# Autodesk Inventor assembly: White Knight
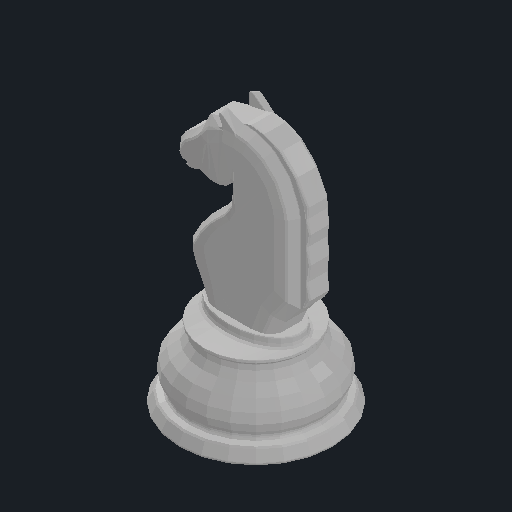
[picture p0: Inventor's stored thumbnail of the model, 512x512]
Saved by Autodesk Inventor 2026 (Build 300175000, 175)
## iProperties
Created: 2025-04-16
Part Number: White Knight
Document SubType Name: Assembly
Designer: ckyiu
Author: ckyiu
## Documents named in this file (3)
- F:\Chessboard-Design\Design\Core\Chess Pieces\Black Knight.iam
- F:\Chessboard-Design\Design\Core\Chess Pieces\Parts\White Knight.ipt
- F:\Chessboard-Design\Design\My-Inventor-Parts\Hardware\(9.5mm diameter 1.6mm height) 5862K143_Neodymium Magnet.ipt
## Components (2 placed, 2 different names)
1. White Knight:1 — Insert:1
2. (9.5mm diameter 1.6mm height) 5862K143_Neodymium Magnet:1 — Insert:1
## Relationships (1: Insert 1)
- Insert:1: White Knight:1 ↔ (9.5mm diameter 1.6mm height) 5862K143_Neodymium Magnet:1
